# Autodesk Inventor assembly: 4PlatesNMiddleShaft
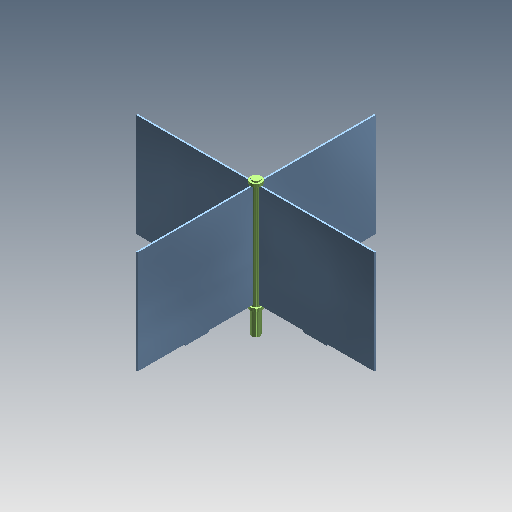
[picture p0: Inventor's stored thumbnail of the model, 512x512]
Saved by Autodesk Inventor 2018 (Build 220112000, 112)
## iProperties
Created: 2017-12-09
Part Number: 4PlatesNMiddleShaft
Document SubType Name: Assembly
Designer: Udara Wanasinghe
Author: Udara Wanasinghe
## Documents named in this file (3)
- D:\Documents\FIT\Hardware Project\Perfect\4PlatesNMiddleShaft.iam
- D:\Documents\FIT\Hardware Project\Perfect\SidePlate.ipt
- D:\Documents\FIT\Hardware Project\Perfect\MiddleShaft.ipt
## Components (5 placed, 2 different names)
1. SidePlate:1 — Rigid:1
2. MiddleShaft:1 — Rigid:1, Rigid:2, Rigid:3, Rigid:4
3. SidePlate:2 — Rigid:2
4. SidePlate:3 — Rigid:4
5. SidePlate:4 — Rigid:3
## Relationships (4: WeldJoint 4)
- Rigid:1 [WeldJoint]: SidePlate:1 ↔ MiddleShaft:1
- Rigid:2 [WeldJoint]: MiddleShaft:1 ↔ SidePlate:2
- Rigid:3 [WeldJoint]: MiddleShaft:1 ↔ SidePlate:4
- Rigid:4 [WeldJoint]: MiddleShaft:1 ↔ SidePlate:3
